# Autodesk Inventor assembly: finalassy
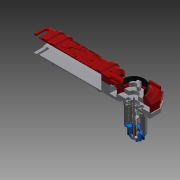
[picture p0: Inventor's stored thumbnail of the model, 180x180]
Saved by Autodesk Inventor 2018 (Build 220112000, 112)
## iProperties
Created: 2019-02-27
Part Number: finalassy
Material: 一般
Document SubType Name: Assembly
Designer: ku_sk
Author: ku_sk
## Documents named in this file (8)
- E:\windows\InventorProjects\BayBladeLauncher\type2\finalassy.iam
- E:\windows\InventorProjects\BayBladeLauncher\type2\parts\bearing.ipt
- E:\windows\InventorProjects\BayBladeLauncher\type2\parts\booledundercover.ipt
- E:\windows\InventorProjects\BayBladeLauncher\type2\parts\conectcover.ipt
- E:\windows\InventorProjects\BayBladeLauncher\type2\parts\uppercover.ipt
- E:\windows\InventorProjects\BayBladeLauncher\type2\parts\topcover.ipt
- E:\windows\InventorProjects\BayBladeLauncher\reedy_540_rc_motor-1.snapshot.2\motor.iam
- E:\windows\InventorProjects\BayBladeLauncher\type2\parts\conecter.ipt
## Components (7 placed, 7 different names)
1. bearing:1 — メイト:4, フラッシュ:1, メイト:16
2. booledundercover:1 — メイト:1, メイト:2, メイト:3, メイト:4, フラッシュ:1, メイト:5, メイト:6, メイト:7, メイト:8, メイト:9, メイト:10, メイト:15, フラッシュ:2
3. uppercover:2 — メイト:8, メイト:9, メイト:10, メイト:11, メイト:12
4. conectcover:1 — メイト:5, メイト:6, メイト:7
5. topcover:1 — メイト:11, メイト:12, メイト:13, メイト:14, メイト:15
6. motor:1 [sub-assembly] — メイト:13, メイト:14
7. conecter:1 — メイト:16, フラッシュ:2
## Relationships (18: Mate 16, Flush 2)
- メイト:1 [Mate]: booledundercover:1
- メイト:2 [Mate]: booledundercover:1
- メイト:3 [Mate]: booledundercover:1
- メイト:4 [Mate]: bearing:1 ↔ booledundercover:1
- フラッシュ:1 [Flush]: bearing:1 ↔ booledundercover:1
- メイト:5 [Mate]: booledundercover:1 ↔ conectcover:1
- メイト:6 [Mate]: booledundercover:1 ↔ conectcover:1
- メイト:7 [Mate]: booledundercover:1 ↔ conectcover:1
- メイト:8 [Mate]: booledundercover:1 ↔ uppercover:2
- メイト:9 [Mate]: booledundercover:1 ↔ uppercover:2
- メイト:10 [Mate]: booledundercover:1 ↔ uppercover:2
- メイト:11 [Mate]: uppercover:2 ↔ topcover:1
- メイト:12 [Mate]: uppercover:2 ↔ topcover:1
- メイト:13 [Mate]: topcover:1 ↔ motor:1
- メイト:14 [Mate]: topcover:1 ↔ motor:1
- メイト:15 [Mate]: booledundercover:1 ↔ topcover:1
- メイト:16 [Mate]: bearing:1 ↔ conecter:1
- フラッシュ:2 [Flush] (11.5 mm): booledundercover:1 ↔ conecter:1
